# Autodesk Inventor assembly: slimV1_mockup
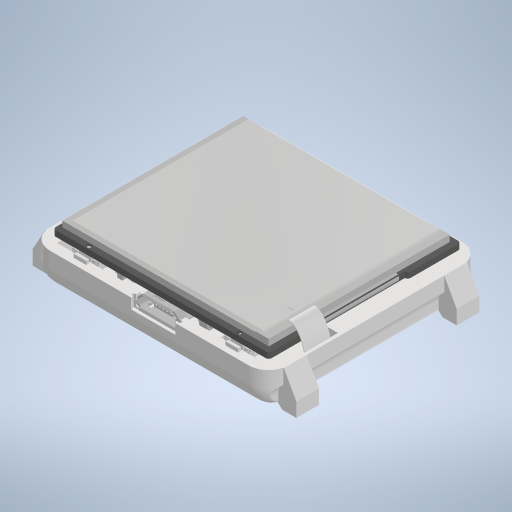
[picture p0: Inventor's stored thumbnail of the model, 512x512]
Saved by Autodesk Inventor 2023 (Build 270158000, 158)
## iProperties
Created: 2023-03-12
Part Number: slimV1_mockup
Document SubType Name: Assembly
Designer: nigel
Author: nigel
## Documents named in this file (3)
- D:\NIGEL\Documents\GitHub\Watchy-CAD\CAD\Cases\SlimTouchscreenV1\slimV1_mockup.iam
- D:\NIGEL\Documents\GitHub\Watchy-CAD\CAD\Cases\SlimTouchscreenV1\SLIM_TC_ASSEMBLED_V1.iam
- D:\NIGEL\Documents\GitHub\Watchy-CAD\CAD\Cases\SlimTouchscreenV1\case_mockup2.ipt
## Components (2 placed, 2 different names)
1. SLIM_TC_ASSEMBLED_V1:1 [sub-assembly] — Flush:1, Mate:1, Flush:2
2. case_mockup2:1 — Flush:1, Mate:1, Flush:2
## Relationships (3: Flush 2, Mate 1)
- Flush:1: SLIM_TC_ASSEMBLED_V1:1 ↔ case_mockup2:1
- Mate:1: SLIM_TC_ASSEMBLED_V1:1 ↔ case_mockup2:1
- Flush:2: SLIM_TC_ASSEMBLED_V1:1 ↔ case_mockup2:1
